# Autodesk Inventor assembly: CollectorHolderAssembly
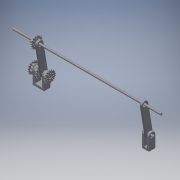
[picture p0: Inventor's stored thumbnail of the model, 180x180]
Saved by Autodesk Inventor 2017 (Build 210142000, 142)
## iProperties
Created: 2017-04-19
Part Number: CollectorHolderAssembly
Document SubType Name: Assembly
Designer: User
Author: User
## Documents named in this file (10)
- C:\Robotics\CAD\2016-17_CAD\CollectorHolderAssembly.iam
- C:\Robotics\CAD\2016-17_CAD\CollectorHolder.ipt
- C:\Robotics\CAD\2016-17_CAD\Axle2.11.ipt
- C:\Robotics\CAD\COTSParts\Actobotics\535 parts\535198.ipt
- C:\Robotics\CAD\COTSParts\Actobotics\545 parts\545556.ipt
- C:\Robotics\CAD\COTSParts\Actobotics\615 parts\615102.ipt
- C:\Robotics\CAD\2016-17_CAD\RollerArm.ipt
- C:\Robotics\CAD\2016-17_CAD\CollecterHolderShort.ipt
- C:\Robotics\CAD\2016-17_CAD\Axle1.34.ipt
- C:\Robotics\CAD\2016-17_CAD\Axle18in.ipt
## Components (20 placed, 9 different names)
1. CollectorHolder:1 — Insert:1, Insert:2, Insert:3, Insert:4, Insert:5, Flush:1, Flush:2
2. Axle2.11:1 — Insert:3
3. 535198:1 — Insert:1, Insert:6
4. 535198:2 — Insert:2, Insert:10
5. 545556:1 — Insert:4, Insert:8
6. 545556:2 — Insert:5, Insert:9
7. 545556:3 — Insert:6, Insert:7
8. 615102:1 — Insert:9
9. 615102:2 — Insert:8
10. 615102:3 — Insert:7
11. RollerArm:1 — Insert:10, Insert:16, Insert:17
12. CollecterHolderShort:1 — Insert:11, Insert:12, Insert:13, Flush:1, Flush:2
13. RollerArm:2 — Insert:14, Insert:15
14. 535198:3 — Insert:11, Insert:14
15. 535198:4 — Insert:12
16. Axle1.34:1 — Insert:13
17. Axle18in:1 — Insert:15, Insert:16
18. 535198:5 — Insert:17, Insert:18
19. 615102:4 — Insert:18, Insert:19
20. 545556:4 — Insert:19
## Relationships (21: Insert 19, Flush 2)
- Insert:1: CollectorHolder:1 ↔ 535198:1
- Insert:2: CollectorHolder:1 ↔ 535198:2
- Insert:3 (-9.779 mm): CollectorHolder:1 ↔ Axle2.11:1
- Insert:4: CollectorHolder:1 ↔ 545556:1
- Insert:5: CollectorHolder:1 ↔ 545556:2
- Insert:6: 535198:1 ↔ 545556:3
- Insert:7: 545556:3 ↔ 615102:3
- Insert:8: 545556:1 ↔ 615102:2
- Insert:9: 545556:2 ↔ 615102:1
- Insert:10: 535198:2 ↔ RollerArm:1
- Insert:11: CollecterHolderShort:1 ↔ 535198:3
- Insert:12: CollecterHolderShort:1 ↔ 535198:4
- Insert:13 (-6.35 mm): CollecterHolderShort:1 ↔ Axle1.34:1
- Insert:14: RollerArm:2 ↔ 535198:3
- Flush:1: CollectorHolder:1 ↔ CollecterHolderShort:1
- Flush:2: CollectorHolder:1 ↔ CollecterHolderShort:1
- Insert:15 (-50.8 mm): RollerArm:2 ↔ Axle18in:1
- Insert:16 (76.2 mm): RollerArm:1 ↔ Axle18in:1
- Insert:17: RollerArm:1 ↔ 535198:5
- Insert:18 (2.667 mm): 535198:5 ↔ 615102:4
- Insert:19: 615102:4 ↔ 545556:4
